# Autodesk Inventor assembly: Slope_testasm
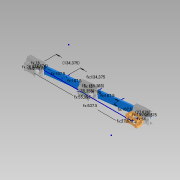
[picture p0: Inventor's stored thumbnail of the model, 180x180]
Saved by Autodesk Inventor 2021 (Build 250183000, 183)
## iProperties
Created: 2021-03-11
Part Number: Slope_testasm
Document SubType Name: Assembly
Designer: kumagai
Author: kumagai
## Documents named in this file (10)
- X:\Develop\CAD\PlaRails\VPUSlope\Slope_testasm.iam
- X:\Develop\CAD\PlaRails\StraightRail\StraightRail_i\StraightMF215.iam
- X:\Develop\CAD\PlaRails\StraightRail\StraightRail_i.iam
- X:\Develop\CAD\PlaRails\VPUSlope\SlopeProfile.ipt
- X:\Develop\CAD\PlaRails\VPUSlope\Slope_HighEnd_C.ipt
- X:\Develop\CAD\PlaRails\ViaductPillarUnit\ViaductPillar_SingleSpan\ViaductPillar_SingleSpan-05u.iam
- X:\Develop\CAD\PlaRails\ViaductPillarUnit\ViaductPillar_SingleSpan.iam
- X:\Develop\CAD\PlaRails\VPUSlope\Slope_Middle_C.ipt
- X:\Develop\CAD\PlaRails\VPUSlope\Slope_LowEndHi.iam
- X:\Develop\CAD\PlaRails\VPUSlope\Slope_LowEndHi\Slope_LowEndHi-FM.iam
## Components (7 placed, 6 different names)
1. Slope_LowEndHi-FM:1 [sub-assembly] — メイト:10, メイト:11
2. Slope_Middle_C:1 — フラッシュ:2, メイト:1, メイト:4, フラッシュ:6, メイト:6, メイト:9, フラッシュ:9
3. StraightMF215:1 [sub-assembly] — メイト:1, メイト:9, フラッシュ:9, メイト:10, メイト:11
4. SlopeProfile:1
5. Slope_HighEnd_C:2 — メイト:7, フラッシュ:7, フラッシュ:8, メイト:8
6. StraightMF215:2 [sub-assembly] — メイト:4, フラッシュ:6, メイト:6, メイト:7
7. ViaductPillar_SingleSpan-05u:1 [sub-assembly] — フラッシュ:7, フラッシュ:8, メイト:8
## Relationships (18: Mate 11, Flush 7)
- フラッシュ:2 [Flush]: Slope_Middle_C:1
- メイト:1 [Mate]: Slope_Middle_C:1 ↔ StraightMF215:1
- [Mate]: Slope_LowEndHi-FM:1 ↔ StraightMF215:1
- [Flush]: Slope_LowEndHi-FM:1 ↔ StraightMF215:1
- [Mate]: Slope_LowEndHi-FM:1 ↔ StraightMF215:1
- [Flush]: Slope_LowEndHi-FM:1 ↔ Slope_HighEnd_C:2
- メイト:4 [Mate]: Slope_Middle_C:1 ↔ StraightMF215:2
- [Mate]: Slope_HighEnd_C:2 ↔ StraightMF215:2
- フラッシュ:6 [Flush]: Slope_Middle_C:1 ↔ StraightMF215:2
- メイト:6 [Mate]: Slope_Middle_C:1 ↔ StraightMF215:2
- メイト:7 [Mate]: Slope_HighEnd_C:2 ↔ StraightMF215:2
- フラッシュ:7 [Flush]: Slope_HighEnd_C:2 ↔ ViaductPillar_SingleSpan-05u:1
- フラッシュ:8 [Flush]: Slope_HighEnd_C:2 ↔ ViaductPillar_SingleSpan-05u:1
- メイト:8 [Mate]: Slope_HighEnd_C:2 ↔ ViaductPillar_SingleSpan-05u:1
- メイト:9 [Mate]: Slope_Middle_C:1 ↔ StraightMF215:1
- フラッシュ:9 [Flush]: Slope_Middle_C:1 ↔ StraightMF215:1
- メイト:10 [Mate]: Slope_LowEndHi-FM:1 ↔ StraightMF215:1
- メイト:11 [Mate]: Slope_LowEndHi-FM:1 ↔ StraightMF215:1
